# Autodesk Inventor assembly: Print_Assembly
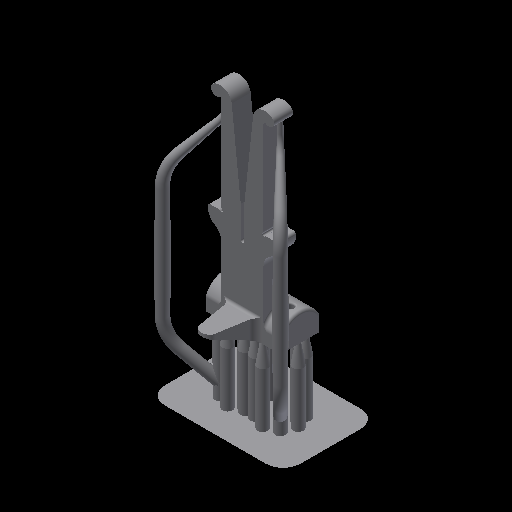
[picture p0: Inventor's stored thumbnail of the model, 512x512]
Saved by Autodesk Inventor 2026.2 (Build 302298010, 298A)
## iProperties
Manager: MANUTENÇÃO GUIFÕES - CP
Company: CP
Created: 2025-09-03
Part Number: Print_Assembly
Project: 0.00 0000/00
Checked By: PMFIGUEIREDO
Engr Approved By: JSSILVA
Description: NOME DA PEÇA/MONTAGEM
Document SubType Name: Assembly
Designer: TPMIRANDA
Engineer: ISO 2768 - m K
Authority: Nº DESENHO PELO QUAL FOI SUBSITUIDO
Stock Number: 00000-000
Title: UME 3400
Subject: CAIXA, INTERIOR, SUPORTE,
Author: TPMIRANDA
Keywords: Caixa de comentários. Substituir texto, ou eliminar.
Comments: UQE2300 UQE2400 UTE2240 UDD9630 CARRUAGENS SIMAFE CARRUAGENS CAF CARRUAGENS ARCO
Revision Number: Nº DESENHO QUE SUBSTITUI
## Documents named in this file (5)
- C:\Users\tpmiranda\OneDrive - Comboios de Portugal EPE\Engate CNMF\Montagem\Print_Assembly_H0_NEM362_Ø2.iam
- C:\Users\tpmiranda\OneDrive - Comboios de Portugal EPE\Engate CNMF\Montagem\Stand.ipt
- C:\Users\tpmiranda\OneDrive - Comboios de Portugal EPE\Engate CNMF\Montagem\Base h0.ipt
- C:\Users\tpmiranda\OneDrive - Comboios de Portugal EPE\Engate CNMF\Montagem\Stand_Branch_H0.ipt
- C:\Users\tpmiranda\OneDrive - Comboios de Portugal EPE\Engate CNMF\Engates\Engate CNMF H0 NEM362 Ø2.ipt
## Components (19 placed, 4 different names)
1. Base h0:1 — Alinhado:13, Alinhado:14, Alinhado:15
2. Engate CNMF H0 NEM362 Ø2:1 — Coincidente:1, Alinhado:4, Coincidente:2, Coincidente:9, Coincidente:10, Transicional:1, Transicional:2
3. Stand_Branch_H0:1 — Ângulo:1, Transicional:1, Coincidente:12
4. Stand_Branch_H0:2 — Ângulo:2, Transicional:2, Coincidente:11
5. Stand:1 — Alinhado:1, Coincidente:9, Alinhado:3, Coincidente:1
6. Stand:2 — Alinhado:5, Coincidente:10, Alinhado:7
7. Stand:3 — Coincidente:12
8. Stand:4
9. Stand:5
10. Stand:6
11. Stand:7
12. Stand:8
13. Stand:9
14. Stand:10
15. Stand:11 — Coincidente:11
16. Stand:12
17. Stand:13
18. Stand:14
19. Stand:15
## Component patterns: (2 elements), (7 elements, first: Stand:2), Componente de padrão 7:2 (7 elements)
## Relationships (18: Flush 8, Mate 6, Angle 2, Transitional 2)
- Alinhado:1 [Flush]: Stand:1
- Coincidente:9 [Mate]: Engate CNMF H0 NEM362 Ø2:1 ↔ Stand:1
- Alinhado:3 [Flush]: Stand:1
- Coincidente:1 [Mate]: Engate CNMF H0 NEM362 Ø2:1 ↔ Stand:1
- Alinhado:4 [Flush]: Engate CNMF H0 NEM362 Ø2:1
- Coincidente:2 [Mate] (-3.5 mm): Engate CNMF H0 NEM362 Ø2:1
- Alinhado:5 [Flush] (2.6 mm): Stand:2
- Coincidente:10 [Mate]: Engate CNMF H0 NEM362 Ø2:1 ↔ Stand:2
- Alinhado:7 [Flush]: Stand:2
- Alinhado:13 [Flush]: Base h0:1
- Ângulo:1 [Angle] (45 deg): Stand_Branch_H0:1
- Ângulo:2 [Angle] (-45 deg): Stand_Branch_H0:2
- Transicional:1: Engate CNMF H0 NEM362 Ø2:1 ↔ Stand_Branch_H0:1
- Alinhado:14 [Flush]: Base h0:1
- Alinhado:15 [Flush] (-3.5 mm): Base h0:1
- Transicional:2: Engate CNMF H0 NEM362 Ø2:1 ↔ Stand_Branch_H0:2
- Coincidente:11 [Mate]: Stand_Branch_H0:2 ↔ Stand:11
- Coincidente:12 [Mate]: Stand_Branch_H0:1 ↔ Stand:3
